# Autodesk Inventor assembly: right_leg
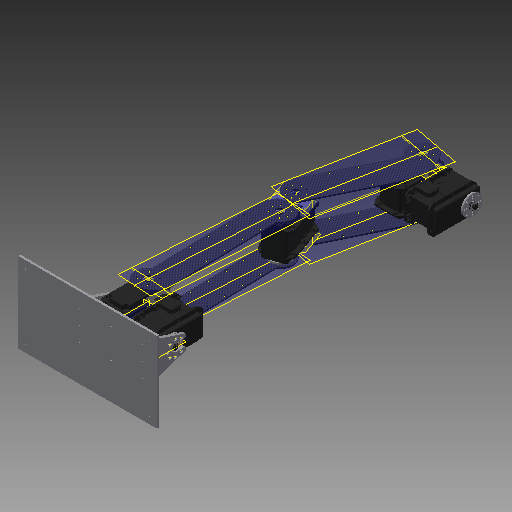
[picture p0: Inventor's stored thumbnail of the model, 512x512]
Saved by Autodesk Inventor 2018 (Build 220112000, 112)
## iProperties
Created: 2018-11-26
Part Number: right_leg
Document SubType Name: Assembly
Designer: bitbots
Mass: 578.907 g
Surface Area: 2185.74 cm^2
Volume: 578.907 cm^3
Density: 1 g/cm^3
Author: bitbots
## Documents named in this file (9)
- C:\Users\bitbots\Desktop\bitbots_hardware\wolfgang\assembly\legs\right_leg.iam
- C:\Users\bitbots\Desktop\bitbots_hardware\wolfgang\assembly\legs\lower_leg.ipt
- C:\Users\bitbots\Desktop\bitbots_hardware\wolfgang\assembly\legs\upper_leg.ipt
- C:\Users\bitbots\Desktop\bitbots_hardware\wolfgang\assembly\motors\MX106\MX-106_with_bearing.iam
- C:\Users\bitbots\Desktop\bitbots_hardware\wolfgang\assembly\legs\knee_connector.ipt
- C:\Users\bitbots\Desktop\bitbots_hardware\wolfgang\assembly\legs\motor_connector.ipt
- C:\Users\bitbots\Desktop\bitbots_hardware\wolfgang\assembly\motors\MX106\MX-106_with_horn.iam
- C:\Users\bitbots\Desktop\bitbots_hardware\wolfgang\assembly\legs\ankle.ipt
- C:\Users\bitbots\Desktop\bitbots_hardware\wolfgang\assembly\legs\foot.ipt
## Components (17 placed, 8 different names)
1. lower_leg:1 — Mate:39, Mate:40, Mate:41, Mate:57, Mate:58
2. upper_leg:1 — Mate:31, Mate:32, Mate:33, Mate:34, Mate:35
3. lower_leg:2 — Mate:61, Mate:64, Mate:80, Mate:81
4. upper_leg:2 — Mate:28, Mate:36, Mate:37, Mate:38, Mate:82
5. MX-106_with_bearing:1 [sub-assembly] — Mate:16, Mate:17, Mate:18, Mate:20, Mate:21, Mate:22, Mate:39, Mate:40, Mate:41, Mate:61, Mate:81
6. MX-106_with_bearing:2 [sub-assembly] — Mate:5, Mate:6, Mate:7, Mate:8, Mate:9, Mate:10, Mate:28, Mate:29, Mate:31, Mate:32, Mate:33, Mate:82
7. knee_connector:1 — Mate:20, Mate:21, Mate:22, Mate:36, Mate:37, Mate:38
8. knee_connector:2 — Mate:16, Mate:17, Mate:18, Mate:34, Mate:35
9. motor_connector:1 — Mate:65, Mate:66, Mate:67, Mate:71
10. motor_connector:2 — Mate:68, Mate:69, Mate:70, Mate:72, Mate:73
11. motor_connector:3 — Mate:8, Mate:9, Mate:10, Mate:11, Mate:12
12. motor_connector:4 — Mate:5, Mate:6, Mate:7, Mate:13
13. MX-106_with_horn:1 [sub-assembly] — Mate:11, Mate:12, Mate:13, Mate:30
14. MX-106_with_bearing:6 [sub-assembly] — Mate:57, Mate:58, Mate:64, Mate:65, Mate:66, Mate:67, Mate:68, Mate:69, Mate:70, Mate:80
15. MX-106_with_horn:2 [sub-assembly] — Mate:71, Mate:72, Mate:73, Mate:74, Mate:75, Mate:76
16. ankle:1 — Mate:74, Mate:75, Mate:76, Mate:77, Mate:78, Mate:79
17. foot:1 — Mate:77, Mate:78, Mate:79, Angle:1
## Relationships (52: Mate 51, Angle 1)
- Mate:5: MX-106_with_bearing:2 ↔ motor_connector:4
- Mate:6: MX-106_with_bearing:2 ↔ motor_connector:4
- Mate:7: MX-106_with_bearing:2 ↔ motor_connector:4
- Mate:8: MX-106_with_bearing:2 ↔ motor_connector:3
- Mate:9: MX-106_with_bearing:2 ↔ motor_connector:3
- Mate:10: MX-106_with_bearing:2 ↔ motor_connector:3
- Mate:11: motor_connector:3 ↔ MX-106_with_horn:1
- Mate:12: motor_connector:3 ↔ MX-106_with_horn:1
- Mate:13: motor_connector:4 ↔ MX-106_with_horn:1
- Mate:16: MX-106_with_bearing:1 ↔ knee_connector:2
- Mate:17: MX-106_with_bearing:1 ↔ knee_connector:2
- Mate:18: MX-106_with_bearing:1 ↔ knee_connector:2
- Mate:20: MX-106_with_bearing:1 ↔ knee_connector:1
- Mate:21: MX-106_with_bearing:1 ↔ knee_connector:1
- Mate:22: MX-106_with_bearing:1 ↔ knee_connector:1
- Mate:28: upper_leg:2 ↔ MX-106_with_bearing:2
- Mate:29: MX-106_with_bearing:2
- Mate:30: MX-106_with_horn:1
- Mate:31: upper_leg:1 ↔ MX-106_with_bearing:2
- Mate:32: upper_leg:1 ↔ MX-106_with_bearing:2
- Mate:33: upper_leg:1 ↔ MX-106_with_bearing:2
- Mate:34: upper_leg:1 ↔ knee_connector:2
- Mate:35: upper_leg:1 ↔ knee_connector:2
- Mate:36: upper_leg:2 ↔ knee_connector:1
- Mate:37: upper_leg:2 ↔ knee_connector:1
- Mate:38 (0.65 mm): upper_leg:2 ↔ knee_connector:1
- Mate:39: lower_leg:1 ↔ MX-106_with_bearing:1
- Mate:40: lower_leg:1 ↔ MX-106_with_bearing:1
- Mate:41: lower_leg:1 ↔ MX-106_with_bearing:1
- Mate:57: lower_leg:1 ↔ MX-106_with_bearing:6
- Mate:58: lower_leg:1 ↔ MX-106_with_bearing:6
- Mate:61: lower_leg:2 ↔ MX-106_with_bearing:1
- Mate:64: lower_leg:2 ↔ MX-106_with_bearing:6
- Mate:65: motor_connector:1 ↔ MX-106_with_bearing:6
- Mate:66: motor_connector:1 ↔ MX-106_with_bearing:6
- Mate:67: motor_connector:1 ↔ MX-106_with_bearing:6
- Mate:68: motor_connector:2 ↔ MX-106_with_bearing:6
- Mate:69: motor_connector:2 ↔ MX-106_with_bearing:6
- Mate:70: motor_connector:2 ↔ MX-106_with_bearing:6
- Mate:71: motor_connector:1 ↔ MX-106_with_horn:2
- Mate:72: motor_connector:2 ↔ MX-106_with_horn:2
- Mate:73: motor_connector:2 ↔ MX-106_with_horn:2
- Mate:74: MX-106_with_horn:2 ↔ ankle:1
- Mate:75: MX-106_with_horn:2 ↔ ankle:1
- Mate:76: MX-106_with_horn:2 ↔ ankle:1
- Mate:77: ankle:1 ↔ foot:1
- Mate:78: ankle:1 ↔ foot:1
- Mate:79: ankle:1 ↔ foot:1
- Mate:80: lower_leg:2 ↔ MX-106_with_bearing:6
- Mate:81: lower_leg:2 ↔ MX-106_with_bearing:1
- Mate:82: upper_leg:2 ↔ MX-106_with_bearing:2
- Angle:1 (0 deg): foot:1
